# Autodesk Inventor assembly: Assembly_neje_slide_y_wellplateholder_20mmrod
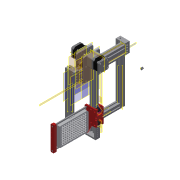
[picture p0: Inventor's stored thumbnail of the model, 180x180]
Saved by Autodesk Inventor 2022 (Build 260153000, 153)
## iProperties
Created: 2021-05-16
Part Number: Assembly_neje_slide_y_wellplateholder_20mmrod
Document SubType Name: Assembly
Designer: diederichbenedict
Mass: 1238.94 g
Surface Area: 8429.73 cm^2
Volume: 1238.94 cm^3
Density: 1 g/cm^3
Author: diederichbenedict
## Documents named in this file (14)
- C:\Users\diederichbenedict\Dropbox\Dokumente\Promotion\PROJECTS\UC2-Hi2\INVENTOR\Assembly_neje_slide_y_wellplateholder_20mmrod.iam
- C:\Users\diederichbenedict\Dropbox\Dokumente\Promotion\PROJECTS\UC2-Hi2\INVENTOR\Assembly_neje_slide_plate.iam
- C:\Users\diederichbenedict\Dropbox\Dokumente\Promotion\PROJECTS\UC2-Hi2\INVENTOR\Neje_Base_Rod_double_20mm.ipt
- C:\Users\diederichbenedict\Dropbox\Dokumente\Promotion\PROJECTS\UC2-Hi2\INVENTOR\10_Base_puzzle_v3.ipt
- C:\Users\diederichbenedict\Dropbox\Dokumente\Promotion\PROJECTS\UC2-Hi2\INVENTOR\Assembly_neje_slide_y_20mmrod.iam
- C:\Users\diederichbenedict\Dropbox\Dokumente\Promotion\PROJECTS\UC2-Hi2\INVENTOR\Neje_Base_Rod_20mm.ipt
- C:\Users\diederichbenedict\Dropbox\Dokumente\Promotion\PROJECTS\UC2-Hi2\INVENTOR\Neje_Base_Rod_20mmX200mm.ipt
- C:\Users\diederichbenedict\Dropbox\Dokumente\Promotion\PROJECTS\UC2-Hi2\INVENTOR\Neje_20mm_rod_connector_double.ipt
- C:\Users\diederichbenedict\Dropbox\Dokumente\Promotion\PROJECTS\UC2-Hi2\INVENTOR\Neje_Endrole_Adapter.ipt
- C:\Users\diederichbenedict\Dropbox\Dokumente\Promotion\PROJECTS\UC2-Hi2\INVENTOR\Neje_20mm_rod_connector_double_R1.ipt
- C:\Users\diederichbenedict\Dropbox\Dokumente\Promotion\PROJECTS\UC2-Hi2\INVENTOR\Neje_distancering.ipt
- C:\Users\diederichbenedict\Dropbox\Dokumente\Promotion\PROJECTS\UC2-Hi2\INVENTOR\00_Gear_Pulley_GT2_nut.ipt
- C:\Users\diederichbenedict\Dropbox\Dokumente\Promotion\PROJECTS\UC2-Hi2\INVENTOR\00_Aluminiumrail_nutslider_block.ipt
- C:\Users\diederichbenedict\Dropbox\Dokumente\Promotion\PROJECTS\UC2-Hi2\INVENTOR\Neje_Rolls_small.ipt
## Components (38 placed, 14 different names)
1. Neje_Base_Rod_double_20mm:1 — Angle:1, Flush:10, Flush:11, Mate:7, Mate:22, Flush:22, Mate:23, Tangent:1, Flush:28, Angle:2, Flush:31, Flush:32, Flush:33, Insert:3
2. Assembly_neje_slide_plate:1 [sub-assembly] — Mate:26, Mate:29, Flush:36, Mate:31
3. Neje_Base_Rod_20mm:2 — Flush:25, Flush:29, Flush:31, Mate:25
4. Neje_Base_Rod_20mm_250mm:5 — Mate:22, Flush:22, Mate:23, Flush:25, Flush:26, Mate:24, Flush:27, Angle:3
5. Neje_Base_Rod_20mmX200mm:1 — Flush:26, Mate:24, Flush:27, Flush:29, Mate:25, Mate:30, Tangent:2, Mate:32, Tangent:3
6. Assembly_neje_slide_y_20mmrod:1 [sub-assembly] — Tangent:1, Flush:28, Angle:2, Mate:26, Flush:34, Flush:35, Mate:29, Flush:36, Flush:37, Flush:38, Flush:39, Insert:4, Insert:5, Insert:6, Insert:7, Insert:8, Mate:33
7. Neje_20mm_rod_connector_double:1 — Flush:32, Flush:33
8. Neje_Endrole_Adapter:1 — Flush:34, Flush:35
9. Neje_20mm_rod_connector_double_R1:1 — Insert:3, Angle:3
10. Neje_distancering:1 — Flush:37, Flush:38, Flush:39
11. Neje_distancering:2 — Insert:6
12. Neje_distancering:3 — Insert:4
13. Neje_distancering:4 — Insert:5
14. 00_Gear_Pulley_GT2_nut:1 — Insert:7
15. 00_Gear_Pulley_GT2_nut:2 — Insert:8
16. 00_Aluminiumrail_nutslider_block:1
17. Neje_Rolls_small:1 — Mate:30, Tangent:2, Mate:31
18. Neje_Rolls_small:2 — Mate:32, Mate:33, Tangent:3
19. 10_Base_puzzle_v3:1 — Flush:10, Flush:11, Mate:7
20. 10_Base_puzzle_v3:2
21. 10_Base_puzzle_v3:3
22. 10_Base_puzzle_v3:4
23. 10_Base_puzzle_v3:5
24. 10_Base_puzzle_v3:6
25. 10_Base_puzzle_v3:7
26. 10_Base_puzzle_v3:8
27. 10_Base_puzzle_v3:9
28. 10_Base_puzzle_v3:10
29. 10_Base_puzzle_v3:11
30. 10_Base_puzzle_v3:12
31. 10_Base_puzzle_v3:13
32. 10_Base_puzzle_v3:14
33. 10_Base_puzzle_v3:15
34. 10_Base_puzzle_v3:16
35. 10_Base_puzzle_v3:17
36. 10_Base_puzzle_v3:18
37. 10_Base_puzzle_v3:19
38. 10_Base_puzzle_v3:20
## Component patterns: (5 elements), (4 elements, first: 10_Base_puzzle_v3:1), Component Pattern 1:2 (4 elements), Component Pattern 1:3 (4 elements), Component Pattern 1:4 (4 elements), Component Pattern 1:5 (4 elements)
## Relationships (40: Flush 17, Mate 11, Insert 6, Angle 3, Tangent 3)
- Angle:1 (180 deg): Neje_Base_Rod_double_20mm:1
- Flush:10 (-80 mm): Neje_Base_Rod_double_20mm:1 ↔ 10_Base_puzzle_v3:1
- Flush:11: Neje_Base_Rod_double_20mm:1 ↔ 10_Base_puzzle_v3:1
- Mate:7 (-15 mm): Neje_Base_Rod_double_20mm:1 ↔ 10_Base_puzzle_v3:1
- Mate:22: Neje_Base_Rod_double_20mm:1 ↔ Neje_Base_Rod_20mm_250mm:5
- Flush:22: Neje_Base_Rod_double_20mm:1 ↔ Neje_Base_Rod_20mm_250mm:5
- Mate:23: Neje_Base_Rod_double_20mm:1 ↔ Neje_Base_Rod_20mm_250mm:5
- Flush:25: Neje_Base_Rod_20mm:2 ↔ Neje_Base_Rod_20mm_250mm:5
- Flush:26: Neje_Base_Rod_20mm_250mm:5 ↔ Neje_Base_Rod_20mmX200mm:1
- Mate:24: Neje_Base_Rod_20mm_250mm:5 ↔ Neje_Base_Rod_20mmX200mm:1
- Flush:27: Neje_Base_Rod_20mm_250mm:5 ↔ Neje_Base_Rod_20mmX200mm:1
- Tangent:1 (-1 mm): Neje_Base_Rod_double_20mm:1 ↔ Assembly_neje_slide_y_20mmrod:1
- Flush:28: Neje_Base_Rod_double_20mm:1 ↔ Assembly_neje_slide_y_20mmrod:1
- Angle:2 (0 deg): Neje_Base_Rod_double_20mm:1 ↔ Assembly_neje_slide_y_20mmrod:1
- Flush:29: Neje_Base_Rod_20mm:2 ↔ Neje_Base_Rod_20mmX200mm:1
- Flush:31: Neje_Base_Rod_double_20mm:1 ↔ Neje_Base_Rod_20mm:2
- Mate:25: Neje_Base_Rod_20mm:2 ↔ Neje_Base_Rod_20mmX200mm:1
- Flush:32: Neje_Base_Rod_double_20mm:1 ↔ Neje_20mm_rod_connector_double:1
- Flush:33: Neje_Base_Rod_double_20mm:1 ↔ Neje_20mm_rod_connector_double:1
- Mate:26: Assembly_neje_slide_plate:1 ↔ Assembly_neje_slide_y_20mmrod:1
- Flush:34: Assembly_neje_slide_y_20mmrod:1 ↔ Neje_Endrole_Adapter:1
- Flush:35: Assembly_neje_slide_y_20mmrod:1 ↔ Neje_Endrole_Adapter:1
- Insert:3: Neje_Base_Rod_double_20mm:1 ↔ Neje_20mm_rod_connector_double_R1:1
- Angle:3 (180 deg): Neje_Base_Rod_20mm_250mm:5 ↔ Neje_20mm_rod_connector_double_R1:1
- Mate:29: Assembly_neje_slide_plate:1 ↔ Assembly_neje_slide_y_20mmrod:1
- Flush:36 (-15 mm): Assembly_neje_slide_plate:1 ↔ Assembly_neje_slide_y_20mmrod:1
- Flush:37: Assembly_neje_slide_y_20mmrod:1 ↔ Neje_distancering:1
- Flush:38: Assembly_neje_slide_y_20mmrod:1 ↔ Neje_distancering:1
- Flush:39: Assembly_neje_slide_y_20mmrod:1 ↔ Neje_distancering:1
- Insert:4: Assembly_neje_slide_y_20mmrod:1 ↔ Neje_distancering:3
- Insert:5: Assembly_neje_slide_y_20mmrod:1 ↔ Neje_distancering:4
- Insert:6: Assembly_neje_slide_y_20mmrod:1 ↔ Neje_distancering:2
- Insert:7: Assembly_neje_slide_y_20mmrod:1 ↔ 00_Gear_Pulley_GT2_nut:1
- Insert:8 (-9 mm): Assembly_neje_slide_y_20mmrod:1 ↔ 00_Gear_Pulley_GT2_nut:2
- Mate:30: Neje_Base_Rod_20mmX200mm:1 ↔ Neje_Rolls_small:1
- Tangent:2 (-0.5 mm): Neje_Base_Rod_20mmX200mm:1 ↔ Neje_Rolls_small:1
- Mate:31: Assembly_neje_slide_plate:1 ↔ Neje_Rolls_small:1
- Mate:32 (1.763 mm): Neje_Base_Rod_20mmX200mm:1 ↔ Neje_Rolls_small:2
- Mate:33: Assembly_neje_slide_y_20mmrod:1 ↔ Neje_Rolls_small:2
- Tangent:3 (-0.5 mm): Neje_Base_Rod_20mmX200mm:1 ↔ Neje_Rolls_small:2
